# Autodesk Inventor assembly: dome with double door
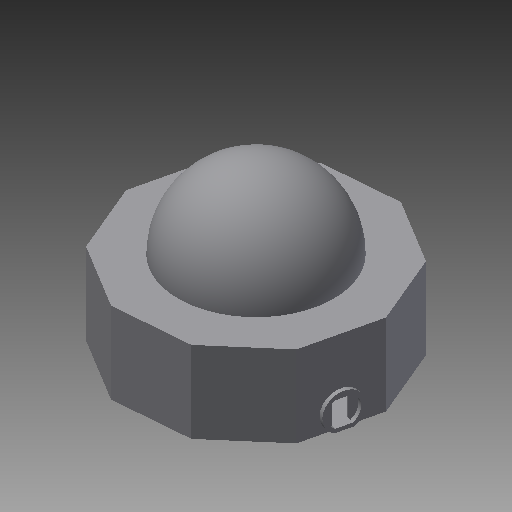
[picture p0: Inventor's stored thumbnail of the model, 512x512]
Saved by Autodesk Inventor 2017 (Build 210142000, 142)
## iProperties
Created: 2018-03-14
Part Number: dome with double door
Document SubType Name: Assembly
Designer: braxtonwright
Author: braxtonwright
## Documents named in this file (3)
- D:\School\Game develpment\geoscape\done\rooms\assembly\dome with double door.iam
- D:\School\Game develpment\geoscape\done\rooms\dome.ipt
- D:\School\Game develpment\geoscape\done\doors\double door.ipt
## Components (3 placed, 3 different names)
1. dome:1 — Mate:1, Mate:2, Mate:3, Mate:4, Flush:1, Flush:2
2. right double door:1 — Mate:1, Mate:4, Flush:1
3. left double door:2 — Mate:2, Mate:3, Flush:2
## Relationships (6: Mate 4, Flush 2)
- Mate:1: dome:1 ↔ right double door:1
- Mate:2: dome:1 ↔ left double door:2
- Mate:3: dome:1 ↔ left double door:2
- Mate:4: dome:1 ↔ right double door:1
- Flush:1: dome:1 ↔ right double door:1
- Flush:2: dome:1 ↔ left double door:2
